# Autodesk Inventor assembly: 1310-0016-4012 assembly
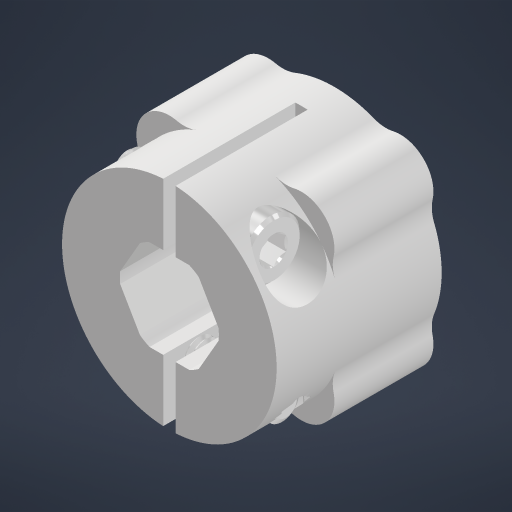
[picture p0: Inventor's stored thumbnail of the model, 512x512]
Saved by Autodesk Inventor 2023 (Build 270158000, 158)
## iProperties
Created: 2018-09-10
Part Number: 1310-0016-4012 assembly
Description: STEP AP203
Document SubType Name: Assembly
Designer: Arash
Title: 1310-0016-4012 assembly.STEP
Revision Number: ANY
Sending System: SolidWorks 2016
Preprocessor: SwSTEP 2.0
## Documents named in this file (3)
- C:\$WorkingFolder\Engineering Data\FTC_Parts_Library\goBilda\Motion\Hubs\Hyper Hubs\Metric (1313 Series)\Hyper Hub (12mm Rex).iam
- C:\$WorkingFolder\Engineering Data\FTC_Parts_Library\goBilda\Motion\Hubs\Hyper Hubs\Metric (1313 Series)\1310-0016-4012.ipt
- C:\$WorkingFolder\Engineering Data\FTC_Parts_Library\ISO Standard Hardware\Screws\Sockethead Screws\Cap Screws\M4 x 0.7mm\(M4 x 0.7 x 14) Sockethead Cap Screw.ipt
## Components (3 placed, 2 different names)
1. 1310-0016-4012_1 — Mate:1, Mate:2, Mate:3, Mate:4
2. (M4 x 0.7 x 14) Sockethead Cap Screw:1 — Mate:1, Mate:2
3. (M4 x 0.7 x 14) Sockethead Cap Screw:2 — Mate:3, Mate:4
## Relationships (4: Mate 4)
- Mate:1: 1310-0016-4012_1 ↔ (M4 x 0.7 x 14) Sockethead Cap Screw:1
- Mate:2: 1310-0016-4012_1 ↔ (M4 x 0.7 x 14) Sockethead Cap Screw:1
- Mate:3: 1310-0016-4012_1 ↔ (M4 x 0.7 x 14) Sockethead Cap Screw:2
- Mate:4: 1310-0016-4012_1 ↔ (M4 x 0.7 x 14) Sockethead Cap Screw:2
